# Autodesk Inventor assembly: Aperatus
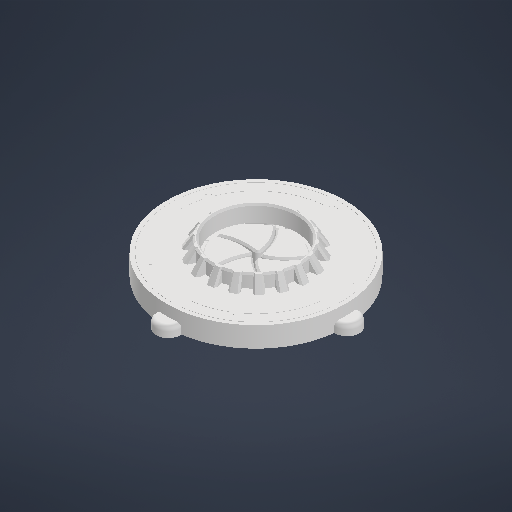
[picture p0: Inventor's stored thumbnail of the model, 512x512]
Saved by Autodesk Inventor 2026.2 (Build 302298000, 298)
## iProperties
Created: 2025-12-30
Part Number: Aperatus
Document SubType Name: Assembly
Designer: Cobble
Author: Cobble
## Documents named in this file (6)
- D:\CAD\Shot FIller V2\Aperatus 100mm\Aperatus.iam
- D:\CAD\Shot FIller V2\Aperatus 100mm\GroundPlate_Aperatus.ipt
- D:\CAD\Shot FIller V2\Aperatus 100mm\Aparatus_Motion_Conveyer.ipt
- D:\CAD\Shot FIller V2\Aperatus 100mm\Aperatus_Blade.ipt
- D:\CAD\Shot FIller V2\Aperatus 100mm\Aparatus_Connector_2.ipt
- D:\CAD\Shot FIller V2\Aperatus 100mm\Aparatus_Motion_Conveyer_Cap.ipt
## Components (13 placed, 5 different names)
1. GroundPlate_Aperatus:1 — Insert:18, Insert:19, Insert:20, Insert:21, Insert:22, Insert:23
2. Aparatus_Motion_Conveyer:1 — Insert:18, Mate:12, Mate:13, Mate:14, Mate:15, Mate:16, Mate:17, Mate:18, Mate:19
3. Aperatus_Blade:1 — Insert:21, Insert:25
4. Aperatus_Blade:2 — Insert:23, Insert:26
5. Aperatus_Blade:3 — Insert:20, Insert:29
6. Aperatus_Blade:4 — Insert:22, Insert:27
7. Aperatus_Blade:5 — Insert:19, Insert:28
8. Aparatus_Motion_Conveyer_Cap:1 — Mate:12, Mate:13, Mate:14
9. Aparatus_Connector_2:3 — Insert:25, Mate:15
10. Aparatus_Connector_2:4 — Mate:16, Insert:26
11. Aparatus_Connector_2:5 — Mate:17, Insert:27
12. Aparatus_Connector_2:6 — Mate:19, Insert:29
13. Aparatus_Connector_2:7 — Mate:18, Insert:28
## Relationships (19: Insert 11, Mate 8)
- Insert:18 (-25 mm): GroundPlate_Aperatus:1 ↔ Aparatus_Motion_Conveyer:1
- Mate:12: Aparatus_Motion_Conveyer:1 ↔ Aparatus_Motion_Conveyer_Cap:1
- Mate:13: Aparatus_Motion_Conveyer:1 ↔ Aparatus_Motion_Conveyer_Cap:1
- Mate:14: Aparatus_Motion_Conveyer:1 ↔ Aparatus_Motion_Conveyer_Cap:1
- Insert:19: GroundPlate_Aperatus:1 ↔ Aperatus_Blade:5
- Insert:20: GroundPlate_Aperatus:1 ↔ Aperatus_Blade:3
- Insert:21: GroundPlate_Aperatus:1 ↔ Aperatus_Blade:1
- Insert:22: GroundPlate_Aperatus:1 ↔ Aperatus_Blade:4
- Insert:23: GroundPlate_Aperatus:1 ↔ Aperatus_Blade:2
- Insert:25: Aperatus_Blade:1 ↔ Aparatus_Connector_2:3
- Mate:15: Aparatus_Motion_Conveyer:1 ↔ Aparatus_Connector_2:3
- Mate:16: Aparatus_Motion_Conveyer:1 ↔ Aparatus_Connector_2:4
- Mate:17: Aparatus_Motion_Conveyer:1 ↔ Aparatus_Connector_2:5
- Mate:18: Aparatus_Motion_Conveyer:1 ↔ Aparatus_Connector_2:7
- Mate:19: Aparatus_Motion_Conveyer:1 ↔ Aparatus_Connector_2:6
- Insert:26: Aperatus_Blade:2 ↔ Aparatus_Connector_2:4
- Insert:27: Aperatus_Blade:4 ↔ Aparatus_Connector_2:5
- Insert:28: Aperatus_Blade:5 ↔ Aparatus_Connector_2:7
- Insert:29: Aperatus_Blade:3 ↔ Aparatus_Connector_2:6
